# Autodesk Inventor assembly: Arm Manipulator
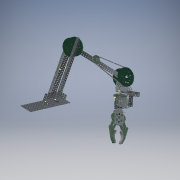
[picture p0: Inventor's stored thumbnail of the model, 180x180]
Saved by Autodesk Inventor 2018 (Build 220112000, 112)
## iProperties
Created: 2018-11-11
Part Number: Arm Manipulator
Document SubType Name: Assembly
Designer: USER
Author: USER
## Documents named in this file (21)
- C:\Users\USER\Desktop\School\Grade 12\Sem 1\Computer Engineering\Competition Robot Inventor\Arm Manipulator.iam
- C:\Users\USER\Downloads\Inventor_2013_VEX_ KOP_-_Metric\Metric\Motion\84 Tooth Gear.ipt
- C:\Users\USER\Downloads\Inventor_2013_VEX_ KOP_-_Metric\Metric\Structure\C-Channel 1x2x1x25 Hole.ipt
- C:\Users\USER\Downloads\Inventor_2013_VEX_ KOP_-_Metric\Metric\Motion\Shaft 4 inch.ipt
- C:\Users\USER\Downloads\Inventor_2013_VEX_ KOP_-_Metric\Metric\Motion\Shaft 3 inch.ipt
- C:\Users\USER\Downloads\Inventor_2013_VEX_ KOP_-_Metric\Metric\Motion\36 Tooth Gear.ipt
- C:\Users\USER\Downloads\Inventor_2013_VEX_ KOP_-_Metric\Metric\Structure\Lin Mot-Rack Brk.ipt
- C:\Users\USER\Downloads\Inventor_2013_VEX_ KOP_-_Metric\Metric\Motion\60 Tooth Gear.ipt
- C:\Users\USER\Downloads\Inventor_2013_VEX_ KOP_-_Metric\Metric\Structure\Pivot Gusset.ipt
- C:\Users\USER\Downloads\Inventor_2013_VEX_ KOP_-_Metric\Metric\Structure\Hinge.iam
- C:\Users\USER\Downloads\Inventor_2013_VEX_ KOP_-_Metric\Metric\Motion\Shaft Collar.iam
- C:\Users\USER\Downloads\Inventor_2013_VEX_ KOP_-_Metric\Metric\Structure\Screw 8-32  x 0.375 inch long.ipt
- C:\Users\USER\Downloads\Inventor_2013_VEX_ KOP_-_Metric\Metric\Motion\Components\VEX Claw Finger.iam
- C:\Users\USER\Downloads\Inventor_2013_VEX_ KOP_-_Metric\Metric\Motion\Components\Gripper_Assembly_SubAssembly.iam
- C:\Users\USER\Downloads\Inventor_2013_VEX_ KOP_-_Metric\Metric\Motion\Components\VEX-12-TOOTH-GEAR.ipt
- C:\Users\USER\Downloads\Inventor_2013_VEX_ KOP_-_Metric\Metric\Motion\Components\Vexplorer-CLAW-GEAR-LINKAGE.ipt
- C:\Users\USER\Downloads\Inventor_2013_VEX_ KOP_-_Metric\Metric\Motion\Components\Vexplorer-CLAW-LINKAGE.ipt
- C:\Users\USER\Downloads\Inventor_2013_VEX_ KOP_-_Metric\Metric\Motion\Components\SHAFT-2000.ipt
- C:\Users\USER\Downloads\Inventor_2013_VEX_ KOP_-_Metric\Metric\Structure\Chassis Bumper 25 Hole.ipt
- C:\Users\USER\Downloads\Inventor_2013_VEX_ KOP_-_Metric\Metric\Structure\Plate 5x25 Hole.ipt
- C:\Users\USER\Downloads\Inventor_2013_VEX_ KOP_-_Metric\Metric\Motion\Chain Link.ipt
## Components (197 placed, 20 different names)
1. 84 Tooth Gear:1 — Rigid:3, Rotational:1, Rigid:11, Rigid:25, Rigid:26
2. 84 Tooth Gear:2 — Rigid:6, Rigid:8
3. 84 Tooth Gear:3 — Rigid:7
4. 84 Tooth Gear:4 — Rigid:2, Rotation:1, Rigid:27, Rigid:28
5. C-Channel 1x2x1x25 Hole:1 — Rotational:1, Rotational:3, Rigid:8, Mate:4, Angle:1
6. Shaft 4 inch:1 — Rigid:3, Rigid:2, Rigid:18, Rigid:19
7. Shaft 4 inch:2 — Rigid:6, Rigid:7, Rigid:21, Rigid:22, Rotational:41
8. Shaft 3 inch:1 — Rotational:3, Rigid:5, Rigid:20, Rigid:31
9. 36 Tooth Gear:1 — Rigid:5, Rotation:1, Flush:1
10. Lin Mot-Rack Brk:1 — Rotational:4, Rigid:11, Rigid:14
11. Lin Mot-Rack Brk:2 — Rigid:10, Rigid:15, Rigid:29, Rigid:30, Rigid:34
12. 60 Tooth Gear:1 — Rigid:9
13. Shaft 3 inch:2 — Rotational:4, Rigid:9, Rigid:10, Rotational:5, Rigid:23, Rigid:24
14. Pivot Gusset:1 — Rigid:15, Rigid:16
15. Pivot Gusset:2 — Rigid:14
16. Hinge:1 [sub-assembly] — Rigid:17
17. Hinge:2 [sub-assembly] — Rigid:16, Rigid:17
18. Shaft Collar:1 [sub-assembly] — Rigid:19
19. Shaft Collar:2 [sub-assembly] — Rigid:20
20. Shaft Collar:3 [sub-assembly] — Rigid:18
21. Shaft Collar:5 [sub-assembly] — Rigid:21
22. Shaft Collar:6 [sub-assembly] — Rotational:5
23. Shaft Collar:7 [sub-assembly] — Rigid:24
24. Shaft Collar:9 [sub-assembly] — Rigid:23
25. Shaft Collar:10 [sub-assembly] — Rigid:22
26. Hexagon Socket Button Head Cap Screw - Inch 8 - 32 x 3/8:1 — Rigid:26
27. Hexagon Socket Button Head Cap Screw - Inch 8 - 32 x 3/8:2 — Rigid:27
28. Hexagon Socket Button Head Cap Screw - Inch 8 - 32 x 3/8:3 — Rigid:25
29. Hexagon Socket Button Head Cap Screw - Inch 8 - 32 x 3/8:4 — Rigid:28
30. Hexagon Socket Button Head Cap Screw - Inch 8 - 32 x 3/8:5 — Rigid:29
31. Hexagon Socket Button Head Cap Screw - Inch 8 - 32 x 3/8:6 — Rigid:30
32. Shaft Collar:11 [sub-assembly] — Rigid:31
33. VEX Claw Finger:1 [sub-assembly] — Rotational:39, Rotational:40
34. VEX Claw Finger:2 [sub-assembly] — Rotational:35, Rotational:36
35. Gripper_Assembly_SubAssembly:1 [sub-assembly] — Rotational:34, Rotational:6, Rotational:7, Rotational:37, Rotational:38, Rigid:34
36. VEX-12-TOOTH-GEAR:1 — Rigid:32, Rotation:2
37. Vexplorer-CLAW-GEAR-LINKAGE:1 — Rotational:37, Rotational:39, Rotation:3
38. Vexplorer-CLAW-LINKAGE:1 — Rotational:38, Rotational:40
39. Vexplorer-CLAW-LINKAGE:2 — Rotational:7, Rotational:36
40. Vexplorer-CLAW-GEAR-LINKAGE:2 — Rotational:6, Rotation:2, Rotational:35, Rotation:3
41. SHAFT-2000:1 — Rigid:32, Rotational:34, Rigid:33
42. Shaft Collar:12 [sub-assembly] — Rigid:33
43. Chassis Bumper 25 Hole:1 — Rigid:41
44. Chassis Bumper 25 Hole:2 — Rotational:41, Rigid:39
45. Plate 5x25 Hole:1 — Rigid:37, Rigid:40
46. Lin Mot-Rack Brk:3 — Rigid:37, Rigid:39
47. Lin Mot-Rack Brk:4 — Rigid:40, Rigid:41
48. Chain Link:1 — Mate:1, Mate:2, Mate:3, Angle:1
49. Chain Link:2
50. Chain Link:3
51. Chain Link:4
52. Chain Link:5
53. Chain Link:6
54. Chain Link:7
55. Chain Link:8
56. Chain Link:9
57. Chain Link:10
58. Chain Link:11
59. Chain Link:12
60. Chain Link:13
61. Chain Link:14
62. Chain Link:15
63. Chain Link:16
64. Chain Link:17
65. Chain Link:18
66. Chain Link:19
67. Chain Link:20
68. Chain Link:21
69. Chain Link:22
70. Chain Link:23
71. Chain Link:24
72. Chain Link:25
73. Chain Link:26
74. Chain Link:27
75. Chain Link:28
76. Chain Link:29
77. Chain Link:30
78. Chain Link:31
79. Chain Link:32
80. Chain Link:33
81. Chain Link:34
82. Chain Link:35
83. Chain Link:36
84. Chain Link:37
85. Chain Link:38
86. Chain Link:39
87. Chain Link:40
88. Chain Link:41
89. Chain Link:42
90. Chain Link:43
91. Chain Link:44
92. Chain Link:45
93. Chain Link:46
94. Chain Link:47
95. Chain Link:48
96. Chain Link:49
97. Chain Link:50
98. Chain Link:51
99. Chain Link:52
100. Chain Link:53
101. Chain Link:54
102. Chain Link:55
103. Chain Link:56
104. Chain Link:57
105. Chain Link:58
106. Chain Link:59
107. Chain Link:60
108. Chain Link:61
109. Chain Link:62
110. Chain Link:63
111. Chain Link:64
112. Chain Link:65
113. Chain Link:66
114. Chain Link:67
115. Chain Link:68
116. Chain Link:69
117. Chain Link:70
118. Chain Link:71
119. Chain Link:72
120. Chain Link:73
121. Chain Link:74
122. Chain Link:75
123. Chain Link:76
124. Chain Link:77
125. Chain Link:78
126. Chain Link:79
127. Chain Link:80
128. Chain Link:81
129. Chain Link:82
130. Chain Link:83
131. Chain Link:84
132. Chain Link:85
133. Chain Link:86
134. Chain Link:87
135. Chain Link:88
136. Chain Link:89
137. Chain Link:90
138. Chain Link:91
139. Chain Link:92
140. Chain Link:93
141. Chain Link:94
142. Chain Link:95
143. Chain Link:96
144. Chain Link:97
145. Chain Link:98
146. Chain Link:99
147. Chain Link:100
148. Chain Link:101
149. Chain Link:102
150. Chain Link:103
151. Chain Link:104
152. Chain Link:105
153. Chain Link:106
154. Chain Link:107
155. Chain Link:108
156. Chain Link:109
157. Chain Link:110
158. Chain Link:111
159. Chain Link:112
160. Chain Link:113
161. Chain Link:114
162. Chain Link:115
163. Chain Link:116
164. Chain Link:117
165. Chain Link:118
166. Chain Link:119
167. Chain Link:120
168. Chain Link:121
169. Chain Link:122
170. Chain Link:123
171. Chain Link:124
172. Chain Link:125
173. Chain Link:126
174. Chain Link:127
175. Chain Link:128
176. Chain Link:129
177. Chain Link:130
178. Chain Link:131
179. Chain Link:132
180. Chain Link:133
181. Chain Link:134
182. Chain Link:135
183. Chain Link:136
184. Chain Link:137
185. Chain Link:138
186. Chain Link:139
187. Chain Link:140
188. Chain Link:141
189. Chain Link:142
190. Chain Link:143
191. Chain Link:144
192. Chain Link:145
193. Chain Link:146
194. Chain Link:147
195. Chain Link:148
196. Chain Link:149
197. Chain Link:150
## Component patterns: (150 elements, first: Chain Link:1)
## Relationships (57: WeldJoint 34, RevoluteJoint 14, Mate 4, RelateRotation 3, Flush 1, Angle 1)
- Rigid:3 [WeldJoint] (25.4 mm): 84 Tooth Gear:1 ↔ Shaft 4 inch:1
- Rigid:2 [WeldJoint] (-38.1 mm): 84 Tooth Gear:4 ↔ Shaft 4 inch:1
- Rotational:1 [RevoluteJoint]: 84 Tooth Gear:1 ↔ C-Channel 1x2x1x25 Hole:1
- Rotational:3 [RevoluteJoint] (-25.4 mm): C-Channel 1x2x1x25 Hole:1 ↔ Shaft 3 inch:1
- Rigid:5 [WeldJoint] (-22.86 mm): Shaft 3 inch:1 ↔ 36 Tooth Gear:1
- Rotation:1 [RelateRotation] (1 ul): 84 Tooth Gear:4 ↔ 36 Tooth Gear:1
- Rigid:6 [WeldJoint] (-31.75 mm): 84 Tooth Gear:2 ↔ Shaft 4 inch:2
- Rigid:7 [WeldJoint] (-25.4 mm): 84 Tooth Gear:3 ↔ Shaft 4 inch:2
- Rigid:8 [WeldJoint] (-6.35 mm): 84 Tooth Gear:2 ↔ C-Channel 1x2x1x25 Hole:1
- Rotational:4 [RevoluteJoint] (-10 mm): Lin Mot-Rack Brk:1 ↔ Shaft 3 inch:2
- Rigid:9 [WeldJoint] (-20 mm): 60 Tooth Gear:1 ↔ Shaft 3 inch:2
- Rigid:10 [WeldJoint] (15 mm): Lin Mot-Rack Brk:2 ↔ Shaft 3 inch:2
- Rigid:11 [WeldJoint]: 84 Tooth Gear:1 ↔ Lin Mot-Rack Brk:1
- Rigid:14 [WeldJoint]: Lin Mot-Rack Brk:1 ↔ Pivot Gusset:2
- Rigid:15 [WeldJoint]: Lin Mot-Rack Brk:2 ↔ Pivot Gusset:1
- Rigid:16 [WeldJoint]: Pivot Gusset:1 ↔ Hinge:2
- Rigid:17 [WeldJoint]: Hinge:1 ↔ Hinge:2
- Rigid:18 [WeldJoint] (-12.7 mm): Shaft 4 inch:1 ↔ Shaft Collar:3
- Rigid:19 [WeldJoint] (-38.1 mm): Shaft 4 inch:1 ↔ Shaft Collar:1
- Rigid:20 [WeldJoint] (-12.7 mm): Shaft 3 inch:1 ↔ Shaft Collar:2
- Rigid:21 [WeldJoint] (-25.4 mm): Shaft 4 inch:2 ↔ Shaft Collar:5
- Rigid:22 [WeldJoint] (-25.4 mm): Shaft 4 inch:2 ↔ Shaft Collar:10
- Rotational:5 [RevoluteJoint] (-3.175 mm): Shaft 3 inch:2 ↔ Shaft Collar:6
- Rigid:23 [WeldJoint] (-9.525 mm): Shaft 3 inch:2 ↔ Shaft Collar:9
- Rigid:24 [WeldJoint] (-14.2875 mm): Shaft 3 inch:2 ↔ Shaft Collar:7
- Rigid:25 [WeldJoint] (-7.9375 mm): 84 Tooth Gear:1 ↔ Hexagon Socket Button Head Cap Screw - Inch 8 - 32 x 3/8:3
- Rigid:26 [WeldJoint] (-9.525 mm): 84 Tooth Gear:1 ↔ Hexagon Socket Button Head Cap Screw - Inch 8 - 32 x 3/8:1
- Rigid:27 [WeldJoint] (-6.35 mm): 84 Tooth Gear:4 ↔ Hexagon Socket Button Head Cap Screw - Inch 8 - 32 x 3/8:2
- Rigid:28 [WeldJoint] (6.35 mm): 84 Tooth Gear:4 ↔ Hexagon Socket Button Head Cap Screw - Inch 8 - 32 x 3/8:4
- Rigid:29 [WeldJoint] (-7.9375 mm): Lin Mot-Rack Brk:2 ↔ Hexagon Socket Button Head Cap Screw - Inch 8 - 32 x 3/8:5
- Rigid:30 [WeldJoint] (-7.9375 mm): Lin Mot-Rack Brk:2 ↔ Hexagon Socket Button Head Cap Screw - Inch 8 - 32 x 3/8:6
- Rigid:31 [WeldJoint] (17.4625 mm): Shaft 3 inch:1 ↔ Shaft Collar:11
- Rigid:32 [WeldJoint] (-20.6375 mm): VEX-12-TOOTH-GEAR:1 ↔ SHAFT-2000:1
- Rotational:34 [RevoluteJoint] (31.75 mm): Gripper_Assembly_SubAssembly:1 ↔ SHAFT-2000:1
- Rotational:6 [RevoluteJoint]: Gripper_Assembly_SubAssembly:1 ↔ Vexplorer-CLAW-GEAR-LINKAGE:2
- Rotation:2 [RelateRotation] (1 ul): VEX-12-TOOTH-GEAR:1 ↔ Vexplorer-CLAW-GEAR-LINKAGE:2
- Rotational:7 [RevoluteJoint]: Gripper_Assembly_SubAssembly:1 ↔ Vexplorer-CLAW-LINKAGE:2
- Rotational:35 [RevoluteJoint]: VEX Claw Finger:2 ↔ Vexplorer-CLAW-GEAR-LINKAGE:2
- Rotational:36 [RevoluteJoint]: VEX Claw Finger:2 ↔ Vexplorer-CLAW-LINKAGE:2
- Rotational:37 [RevoluteJoint]: Gripper_Assembly_SubAssembly:1 ↔ Vexplorer-CLAW-GEAR-LINKAGE:1
- Rotational:38 [RevoluteJoint]: Gripper_Assembly_SubAssembly:1 ↔ Vexplorer-CLAW-LINKAGE:1
- Rotational:39 [RevoluteJoint]: VEX Claw Finger:1 ↔ Vexplorer-CLAW-GEAR-LINKAGE:1
- Rotational:40 [RevoluteJoint]: VEX Claw Finger:1 ↔ Vexplorer-CLAW-LINKAGE:1
- Rigid:33 [WeldJoint] (-17.4625 mm): SHAFT-2000:1 ↔ Shaft Collar:12
- Rigid:34 [WeldJoint]: Lin Mot-Rack Brk:2 ↔ Gripper_Assembly_SubAssembly:1
- Rotation:3 [RelateRotation] (1 ul): Vexplorer-CLAW-GEAR-LINKAGE:1 ↔ Vexplorer-CLAW-GEAR-LINKAGE:2
- Rotational:41 [RevoluteJoint] (25.4 mm): Shaft 4 inch:2 ↔ Chassis Bumper 25 Hole:2
- Rigid:37 [WeldJoint]: Plate 5x25 Hole:1 ↔ Lin Mot-Rack Brk:3
- Rigid:39 [WeldJoint]: Chassis Bumper 25 Hole:2 ↔ Lin Mot-Rack Brk:3
- Rigid:40 [WeldJoint]: Plate 5x25 Hole:1 ↔ Lin Mot-Rack Brk:4
- Rigid:41 [WeldJoint]: Chassis Bumper 25 Hole:1 ↔ Lin Mot-Rack Brk:4
- Flush:1 (-3.81 mm): 36 Tooth Gear:1
- Mate:1: Chain Link:1
- Mate:2: Chain Link:1
- Mate:3: Chain Link:1
- Mate:4: C-Channel 1x2x1x25 Hole:1
- Angle:1 (-90 deg): C-Channel 1x2x1x25 Hole:1 ↔ Chain Link:1
